# Autodesk Inventor assembly: Wrist
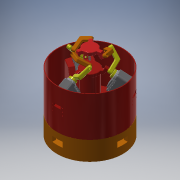
[picture p0: Inventor's stored thumbnail of the model, 180x180]
Saved by Autodesk Inventor 2019 (Build 230136000, 136)
## iProperties
Created: 2022-08-01
Part Number: Wrist
Document SubType Name: Assembly
Designer: zreik
Author: zreik
## Documents named in this file (3)
- D:\Documents\HIAST\4th year\4th Year Project\Design\DirectConnection\Wrist.iam
- D:\Documents\HIAST\4th year\4th Year Project\Design\DirectConnection\SPM.iam
- D:\Documents\HIAST\4th year\4th Year Project\Design\DirectConnection\Base.ipt
## Components (2 placed, 2 different names)
1. SPM:1 [sub-assembly] — Mate:1, Mate:3, Mate:6, Mate:7
2. Base:1 — Mate:1, Mate:3, Mate:4, Flush:1, Mate:5, Mate:6, Mate:7
## Relationships (7: Mate 6, Flush 1)
- Mate:1: SPM:1 ↔ Base:1
- Mate:3: SPM:1 ↔ Base:1
- Mate:4: Base:1
- Flush:1: Base:1
- Mate:5: Base:1
- Mate:6: SPM:1 ↔ Base:1
- Mate:7: SPM:1 ↔ Base:1
